# Autodesk Inventor assembly: SmallSize(2xl)
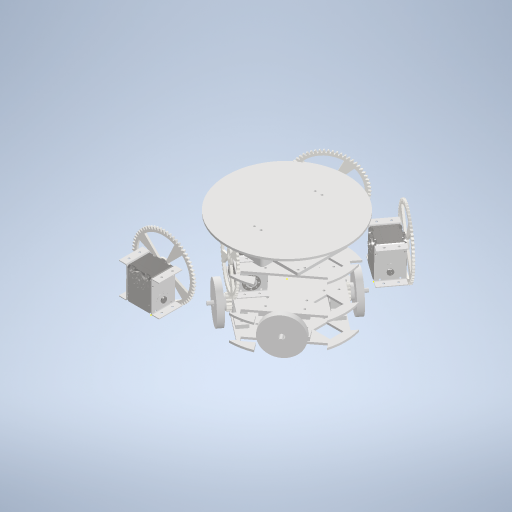
[picture p0: Inventor's stored thumbnail of the model, 512x512]
Saved by Autodesk Inventor 2023 (Build 270158000, 158)
## iProperties
Created: 2022-09-08
Part Number: SmallSize(2xl)
Document SubType Name: Assembly
Designer: Lab. de Manufactura
Author: Lab. de Manufactura
## Documents named in this file (7)
- C:\Users\hiago.sodre\Downloads\SSLurubots\SmallSize(2xl).iam
- C:\Users\hiago.sodre\Downloads\SSLurubots\newbase.ipt
- C:\Users\hiago.sodre\Downloads\SSLurubots\soporte_eje_omni.ipt
- C:\Users\hiago.sodre\Downloads\SSLurubots\EjeRueda.iam
- C:\Users\hiago.sodre\Downloads\SSLurubots\pablo opencr.ipt
- C:\Users\hiago.sodre\Downloads\SSLurubots\hiago_tampassl2.ipt
- C:\Users\hiago.sodre\Downloads\SSLurubots\2XL-430montado.iam
## Components (17 placed, 6 different names)
1. newbase:1 — Rígido:8, Rígido:9, Rígido:10, Rígido:16
2. soporte_eje_omni:1 — Rígido:16, Rígido:17, Rígido:18
3. soporte_eje_omni:2 — Rígido:8, Rígido:19
4. soporte_eje_omni:3 — Rígido:10, Rígido:20
5. soporte_eje_omni:4 — Rígido:9, De rotación:1
6. newbase:2 — Rígido:17, Mate:3
7. newbase:3 — Mate:1
8. EjeRueda:1 [sub-assembly] — De rotación:1
9. EjeRueda:2 [sub-assembly] — Rígido:18
10. EjeRueda:3 [sub-assembly] — Rígido:19
11. EjeRueda:4 [sub-assembly] — Rígido:20
12. pablo opencr:1 — Mate:1, Mate:2
13. hiago_tampassl2:1 — Mate:2
14. 2XL-430montado:1 [sub-assembly]
15. 2XL-430montado:3 [sub-assembly]
16. 2XL-430montado:4 [sub-assembly] — Mate:3
17. 2XL-430montado:5 [sub-assembly]
## Relationships (12: WeldJoint 8, Mate 3, RevoluteJoint 1)
- Rígido:8 [WeldJoint]: newbase:1 ↔ soporte_eje_omni:2
- Rígido:9 [WeldJoint]: newbase:1 ↔ soporte_eje_omni:4
- Rígido:10 [WeldJoint]: newbase:1 ↔ soporte_eje_omni:3
- Rígido:16 [WeldJoint]: newbase:1 ↔ soporte_eje_omni:1
- Rígido:17 [WeldJoint]: soporte_eje_omni:1 ↔ newbase:2
- Rígido:18 [WeldJoint]: soporte_eje_omni:1 ↔ EjeRueda:2
- Rígido:19 [WeldJoint]: soporte_eje_omni:2 ↔ EjeRueda:3
- Rígido:20 [WeldJoint]: soporte_eje_omni:3 ↔ EjeRueda:4
- De rotación:1 [RevoluteJoint]: soporte_eje_omni:4 ↔ EjeRueda:1
- Mate:1: newbase:3 ↔ pablo opencr:1
- Mate:2: pablo opencr:1 ↔ hiago_tampassl2:1
- Mate:3: newbase:2 ↔ 2XL-430montado:4
